# Autodesk Inventor assembly: DetectionRegionRender1
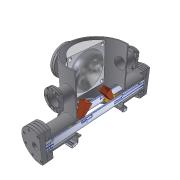
[picture p0: Inventor's stored thumbnail of the model, 180x180]
Saved by Autodesk Inventor 2015 SP1 (Build 190203100, 203)
## iProperties
Created: 2016-07-28
Part Number: DetectionRegionRender1
Document SubType Name: Assembly
Designer: I Rabey
Author: I Rabey
## Documents named in this file (5)
- C:\ColdMatter\CADFiles\EDM Machine\Detection Region\DetectionRegionRender1.iam
- C:\ColdMatter\CADFiles\EDM Machine\Detection Region\Detection Region Chamber.iam
- C:\ColdMatter\CADFiles\EDM Machine\Detection Region\Microwave Horn Assembly\Assembled Horns.iam
- C:\ColdMatter\CADFiles\EDM Machine\Detection Region\Re-entrant Flange and Mirrors\Optics Assembly Lens.iam
- C:\ColdMatter\CADFiles\EDM Machine\Detection Region\Microwave Transmission line\DN63CF blank.ipt
## Components (4 placed, 4 different names)
1. Detection Region Chamber:1 [sub-assembly] — Mate:2, Mate:3, Mate:4, Mate:5, Mate:6, Mate:8, Mate:9, Mate:10, Mate:11, Mate:12
2. Assembled Horns:1 [sub-assembly] — Mate:5, Mate:6
3. Optics Assembly Lens:1 [sub-assembly] — Mate:7, Mate:8, Mate:9
4. DN63CF blank:1 — Mate:10, Mate:11, Mate:12
## Relationships (13: Mate 11, Flush 2)
- Mate:2: Detection Region Chamber:1
- Mate:3: Detection Region Chamber:1
- Mate:4: Detection Region Chamber:1
- Mate:5: Detection Region Chamber:1 ↔ Assembled Horns:1
- Mate:6: Detection Region Chamber:1 ↔ Assembled Horns:1
- Mate:7: Optics Assembly Lens:1
- Mate:8: Detection Region Chamber:1 ↔ Optics Assembly Lens:1
- Mate:9: Detection Region Chamber:1 ↔ Optics Assembly Lens:1
- Flush:1 (23 mm)
- Flush:2 (240 mm)
- Mate:10: Detection Region Chamber:1 ↔ DN63CF blank:1
- Mate:11: Detection Region Chamber:1 ↔ DN63CF blank:1
- Mate:12: Detection Region Chamber:1 ↔ DN63CF blank:1
